# Autodesk Inventor assembly: SERVO MOTOR
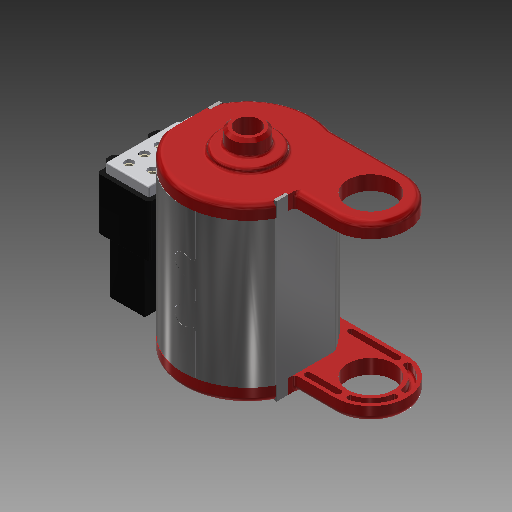
[picture p0: Inventor's stored thumbnail of the model, 512x512]
Saved by Autodesk Inventor 2019 (Build 230136000, 136)
## iProperties
Company: Autodesk Inc.
Created: 2007-10-30
Part Number: SERVO MOTOR
Document SubType Name: Assembly
Designer: Autodesk Inc.
Mass: 92.4419 g
Surface Area: 414.624 cm^2
Volume: 40.6939 cm^3
Density: 2.27164 g/cm^3
Description: SERVO MOTOR 1000
Component Category: Electrical
Author: Inventor
## Documents named in this file (6)
- C:\TEMP\Car Seat\Workspace\Motor.iam
- C:\TEMP\Car Seat\Workspace\Motor Casing.ipt
- C:\TEMP\Car Seat\Workspace\Motor Connector.ipt
- C:\TEMP\Car Seat\Workspace\Motor Endcap L.ipt
- C:\TEMP\Car Seat\Workspace\Motor Endcap R.ipt
- C:\TEMP\Car Seat\Workspace\Motor Connector Plug.ipt
## Components (5 placed, 5 different names)
1. Motor Casing:1
2. Motor Connector:1 — Mate:9, Mate:10, Mate:11
3. Motor Endcap L:1
4. Motor Endcap R:1
5. Motor Connector Plug:1 — Mate:9, Mate:10, Mate:11
## Relationships (12: Mate 11, Flush 1)
- [Mate]: Motor Casing:1 ↔ Motor Connector:1
- [Flush]: Motor Casing:1 ↔ Motor Connector:1
- [Mate]: Motor Casing:1 ↔ Motor Connector:1
- [Mate]: Motor Casing:1 ↔ Motor Endcap L:1
- [Mate]: Motor Casing:1 ↔ Motor Endcap L:1
- [Mate]: Motor Casing:1 ↔ Motor Endcap L:1
- [Mate]: Motor Casing:1 ↔ Motor Endcap R:1
- [Mate]: Motor Casing:1 ↔ Motor Endcap R:1
- [Mate]: Motor Casing:1 ↔ Motor Endcap R:1
- Mate:9: Motor Connector:1 ↔ Motor Connector Plug:1
- Mate:10: Motor Connector:1 ↔ Motor Connector Plug:1
- Mate:11: Motor Connector:1 ↔ Motor Connector Plug:1
